# Autodesk Inventor assembly: Ensamblaje_engranes
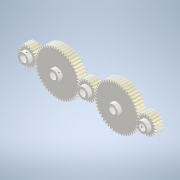
[picture p0: Inventor's stored thumbnail of the model, 180x180]
Saved by Autodesk Inventor 2021 (Build 250183000, 183)
## iProperties
Created: 2021-02-06
Part Number: Ensamblaje_engranes
Document SubType Name: Assembly
Designer: rotje
Author: rotje
## Documents named in this file (3)
- C:\Users\rotje\Documents\Inventor\MSF\Ensamblaje_engranes.iam
- C:\Users\rotje\Documents\Inventor\MSF\Engranaje recto_20_Dientes.ipt
- C:\Users\rotje\Documents\Inventor\MSF\Engranaje recto_50_Dientes.ipt
## Components (5 placed, 2 different names)
1. Engranaje recto1:1 — Coincidencia:1, Coincidencia:2, Tangente:1
2. Engranaje recto2:1 — Coincidencia:3, Tangente:1, Tangente:2, Coincidencia:8
3. Engranaje recto1:3 — Coincidencia:4, Tangente:2, Tangente:3, Coincidencia:9
4. Engranaje recto2:2 — Coincidencia:7, Tangente:3, Tangente:4, Coincidencia:10
5. Engranaje recto1:2 — Coincidencia:6, Tangente:4, Coincidencia:11
## Relationships (14: Mate 10, Tangent 4)
- Coincidencia:1 [Mate]: Engranaje recto1:1
- Coincidencia:2 [Mate]: Engranaje recto1:1
- Coincidencia:3 [Mate]: Engranaje recto2:1
- Coincidencia:4 [Mate]: Engranaje recto1:3
- Coincidencia:6 [Mate]: Engranaje recto1:2
- Coincidencia:7 [Mate]: Engranaje recto2:2
- Tangente:1: Engranaje recto1:1 ↔ Engranaje recto2:1
- Tangente:2: Engranaje recto2:1 ↔ Engranaje recto1:3
- Tangente:3: Engranaje recto1:3 ↔ Engranaje recto2:2
- Tangente:4: Engranaje recto2:2 ↔ Engranaje recto1:2
- Coincidencia:8 [Mate]: Engranaje recto2:1
- Coincidencia:9 [Mate]: Engranaje recto1:3
- Coincidencia:10 [Mate]: Engranaje recto2:2
- Coincidencia:11 [Mate]: Engranaje recto1:2
